# Autodesk Inventor assembly: elevation_assembly
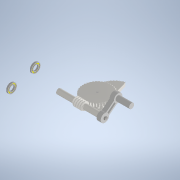
[picture p0: Inventor's stored thumbnail of the model, 180x180]
Saved by Autodesk Inventor 2020 (Build 240168000, 168)
## iProperties
Created: 2020-05-17
Part Number: elevation_assembly
Document SubType Name: Assembly
Designer: Hesekiel
Author: Hesekiel
## Documents named in this file (6)
- C:\Users\Hesekiel\Desktop\Equatorial-Mount-MUM\Mechanika\Mechanizm elewacji Filip\CAD\elevation_assembly.iam
- C:\Users\Hesekiel\Desktop\Equatorial-Mount-MUM\Mechanika\Mechanizm elewacji Filip\CAD\worm_gear.iam
- C:\Users\Hesekiel\Desktop\Equatorial-Mount-MUM\Mechanika\Mechanizm elewacji Filip\CAD\rack_and_pinion.iam
- C:\Users\Hesekiel\Desktop\Equatorial-Mount-MUM\Mechanika\Mechanizm elewacji Filip\CAD\wał_uzębienia.ipt
- C:\Users\Hesekiel\Desktop\Equatorial-Mount-MUM\Mechanika\Mechanizm elewacji Filip\CAD\M6x6_DIN914.ipt
- C:\Users\Hesekiel\Desktop\Equatorial-Mount-MUM\Mechanika\Mechanizm elewacji Filip\CAD\SKF 16006\16006.iam
## Components (7 placed, 5 different names)
1. worm_gear:1 [sub-assembly] — Mate:1, Mate:2, Rotational:4, Angle:1
2. rack_and_pinion:1 [sub-assembly] — Mate:3, Flush:1, Mate:4
3. wał_uzębienia:1 — Mate:1, Mate:2, Rotational:4, Rigid:1, Mate:3, Flush:1, Mate:4, Rigid:2
4. M6x6_DIN914:1 — Rigid:1
5. M6x6_DIN914:2 — Rigid:2
6. 16006:1 [sub-assembly]
7. 16006:2 [sub-assembly]
## Relationships (9: Mate 4, WeldJoint 2, RevoluteJoint 1, Flush 1, Angle 1)
- Mate:1: worm_gear:1 ↔ wał_uzębienia:1
- Mate:2: worm_gear:1 ↔ wał_uzębienia:1
- Rotational:4 [RevoluteJoint]: worm_gear:1 ↔ wał_uzębienia:1
- Rigid:1 [WeldJoint]: wał_uzębienia:1 ↔ M6x6_DIN914:1
- Mate:3: rack_and_pinion:1 ↔ wał_uzębienia:1
- Flush:1: rack_and_pinion:1 ↔ wał_uzębienia:1
- Mate:4: rack_and_pinion:1 ↔ wał_uzębienia:1
- Angle:1 (0 deg): worm_gear:1
- Rigid:2 [WeldJoint]: wał_uzębienia:1 ↔ M6x6_DIN914:2
